# Autodesk Inventor assembly: bubble-wall-v2
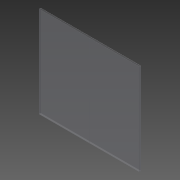
[picture p0: Inventor's stored thumbnail of the model, 180x180]
Saved by Autodesk Inventor 2013 (Build 170138000, 138)
## iProperties
Created: 2013-04-25
Part Number: bubble-wall-v2
Document SubType Name: Assembly
Designer: Chris
Author: Chris
## Documents named in this file (3)
- C:\Users\Chris\Documents\Inventor\Redbull-2013\bubble-wall-v2\bubble-wall-v2.iam
- C:\Users\Chris\Documents\Inventor\Redbull-2013\bubble-wall-v2\bottom.ipt
- C:\Users\Chris\Documents\Inventor\Redbull-2013\bubble-wall-v2\top.ipt
## Components (2 placed, 2 different names)
1. bottom:1 — Flush:1, Mate:1, Flush:2
2. top:1 — Flush:1, Mate:1, Flush:2
## Relationships (3: Flush 2, Mate 1)
- Flush:1: bottom:1 ↔ top:1
- Mate:1: bottom:1 ↔ top:1
- Flush:2: bottom:1 ↔ top:1
